# Autodesk Inventor assembly: Tubo auxiliar 2
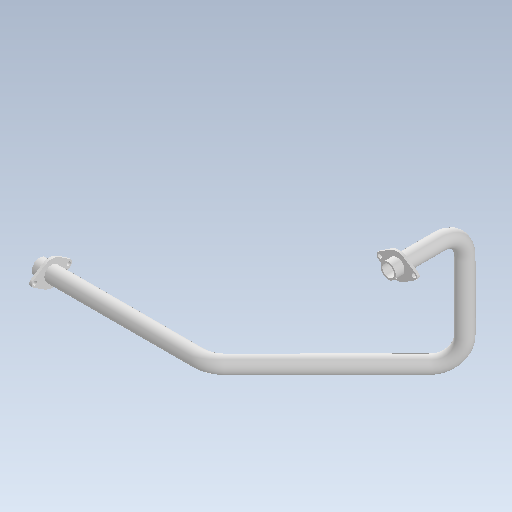
[picture p0: Inventor's stored thumbnail of the model, 512x512]
Saved by Autodesk Inventor 2021 (Build 250183000, 183)
## iProperties
Category: 10
Created: 2021-07-23
Document SubType Name: Assembly
Designer: Giovanni
User Status: 1:4
Author: Giovanni
Keywords: 10
## Documents named in this file (3)
- C:\Users\irineu\Documents\Inventor\MotorRadial7\Tubo auxiliar 2.iam
- C:\Users\irineu\Documents\Inventor\MotorRadial7\Peça25.ipt
- C:\Users\irineu\Documents\Inventor\MotorRadial7\Peça27.ipt
## Components (3 placed, 2 different names)
1. Peça25:1 — Coincidente:1, Alinhado:1, Coincidente:3, Alinhado:2
2. Peça27:1 — Coincidente:3, Alinhado:2, Ângulo:1
3. Peça27:2 — Coincidente:1, Coincidente:2, Alinhado:1
## Relationships (6: Mate 3, Flush 2, Angle 1)
- Coincidente:1 [Mate]: Peça25:1 ↔ Peça27:2
- Coincidente:2 [Mate]: Peça27:2
- Alinhado:1 [Flush] (10 mm): Peça25:1 ↔ Peça27:2
- Coincidente:3 [Mate]: Peça25:1 ↔ Peça27:1
- Alinhado:2 [Flush] (11.62 mm): Peça25:1 ↔ Peça27:1
- Ângulo:1 [Angle] (0 deg): Peça27:1
